# Autodesk Inventor assembly: a
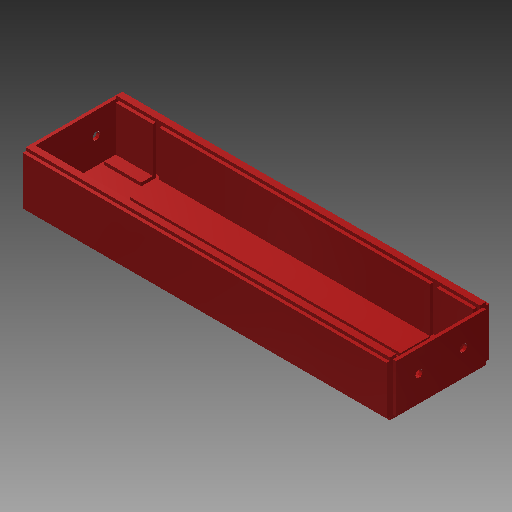
[picture p0: Inventor's stored thumbnail of the model, 512x512]
Saved by Autodesk Inventor 2017 (Build 210142000, 142)
## iProperties
Created: 2015-10-11
Part Number: a
Document SubType Name: Assembly
Designer: daniel
Author: daniel
## Documents named in this file (12)
- C:\Users\daniel\Documents\GitHub\cardboard-stage-metric\stage\a.iam
- C:\Users\daniel\Documents\GitHub\cardboard-stage-metric\stage\aa.ipt
- C:\Users\daniel\Documents\GitHub\cardboard-stage-metric\stage\ab.ipt
- C:\Users\daniel\Documents\GitHub\cardboard-stage-metric\stage\ac.ipt
- C:\Users\daniel\Documents\GitHub\cardboard-stage-metric\stage\ad.ipt
- C:\Users\daniel\Documents\GitHub\cardboard-stage-metric\stage\ae.ipt
- C:\Users\daniel\Documents\GitHub\cardboard-stage-metric\stage\af.ipt
- C:\Users\daniel\Documents\GitHub\cardboard-stage-metric\stage\ah.ipt
- C:\Users\daniel\Documents\GitHub\cardboard-stage-metric\stage\ai.ipt
- C:\Users\daniel\Documents\GitHub\cardboard-stage-metric\stage\base.ipt
- C:\Users\daniel\Documents\GitHub\cardboard-stage-metric\stage\aj.ipt
- C:\Users\daniel\Documents\GitHub\cardboard-stage-metric\stage\ak.ipt
## Components (23 placed, 10 different names)
1. aa:1 — Mate:5, Mate:6, Flush:1, Flush:2, Mate:7, Mate:8, Flush:4, Mate:21, Mate:22, Mate:23
2. ab:1 — Flush:19, Flush:20, Mate:21, Mate:22
3. ac:1 — Flush:19, Flush:20, Mate:23, Mate:24, Flush:24, Mate:26
4. ad:1 — Mate:5, Mate:6, Flush:1, Mate:9, Mate:10, Mate:15
5. ae:1 — Flush:3, Mate:9, Mate:10, Flush:4, Flush:5, Mate:19
6. af:1 — Mate:16, Flush:12, Flush:16, Mate:19, Flush:33, Flush:38, Flush:44, Flush:45
7. ah:1 — Mate:16, Flush:12, Flush:34, Flush:36, Flush:38
8. ad:2 — Flush:2, Mate:7, Mate:8, Mate:11, Flush:7, Flush:37
9. ae:2 — Flush:3, Flush:5, Mate:11, Mate:18, Mate:20, Flush:18
10. ai:1 — Flush:6, Flush:7, Mate:24, Flush:26
11. ai:2 — Flush:6, Mate:15, Mate:25, Flush:23, Flush:24, Flush:25, Mate:26
12. af:2 — Flush:16, Mate:18, Mate:20, Flush:18, Flush:32, Flush:46
13. ah:2 — Flush:36, Flush:47
14. ai:3 — Flush:21, Flush:22, Mate:25, Flush:26
15. ai:4 — Flush:21, Flush:22, Flush:23, Flush:25
16. af:3 — Flush:33
17. ah:3 — Flush:34, Flush:35, Flush:48, Mate:30
18. af:4 — Flush:32
19. ah:4 — Flush:35, Flush:37
20. aj:1 — Flush:39, Flush:42, Flush:43, Flush:46
21. ak:1 — Flush:42, Flush:43, Flush:47, Flush:49
22. aj:2 — Flush:39, Flush:41, Flush:44, Flush:45, Mate:29
23. ak:2 — Flush:41, Mate:29, Flush:48, Mate:30, Flush:49
## Relationships (65: Flush 42, Mate 23)
- Mate:5: aa:1 ↔ ad:1
- Mate:6: aa:1 ↔ ad:1
- Flush:1: aa:1 ↔ ad:1
- Flush:2: aa:1 ↔ ad:2
- Mate:7: aa:1 ↔ ad:2
- Mate:8: aa:1 ↔ ad:2
- Flush:3: ae:1 ↔ ae:2
- Mate:9: ad:1 ↔ ae:1
- Mate:10: ad:1 ↔ ae:1
- Flush:4: aa:1 ↔ ae:1
- Flush:5: ae:1 ↔ ae:2
- Mate:11: ad:2 ↔ ae:2
- Flush:6: ai:1 ↔ ai:2
- Flush:7: ad:2 ↔ ai:1
- Mate:15: ad:1 ↔ ai:2
- Mate:16: af:1 ↔ ah:1
- Flush:12: af:1 ↔ ah:1
- [Mate]: af:2 ↔ ah:2
- [Flush]: af:2 ↔ ah:2
- [Flush]: af:2 ↔ ah:2
- Flush:16: af:1 ↔ af:2
- Mate:19: ae:1 ↔ af:1
- Mate:18: ae:2 ↔ af:2
- Mate:20: ae:2 ↔ af:2
- Flush:18 (-4.3 mm): ae:2 ↔ af:2
- Flush:19: ab:1 ↔ ac:1
- Flush:20: ab:1 ↔ ac:1
- Mate:21: aa:1 ↔ ab:1
- Mate:22: aa:1 ↔ ab:1
- Mate:23: aa:1 ↔ ac:1
- Mate:24: ac:1 ↔ ai:1
- Flush:21: ai:3 ↔ ai:4
- Flush:22: ai:3 ↔ ai:4
- Mate:25: ai:2 ↔ ai:3
- Flush:23: ai:2 ↔ ai:4
- Flush:24: ac:1 ↔ ai:2
- Flush:25: ai:2 ↔ ai:4
- Flush:26: ai:1 ↔ ai:3
- Mate:26: ac:1 ↔ ai:2
- [Mate]: af:3 ↔ ah:3
- [Flush]: af:3 ↔ ah:3
- [Flush]: af:3 ↔ ah:3
- [Mate]: af:4 ↔ ah:4
- [Flush]: af:4 ↔ ah:4
- [Flush]: af:4 ↔ ah:4
- [Flush]: af:3 ↔ af:4
- Flush:32: af:2 ↔ af:4
- Flush:33: af:1 ↔ af:3
- Flush:34: ah:1 ↔ ah:3
- Flush:35: ah:3 ↔ ah:4
- Flush:36: ah:1 ↔ ah:2
- Flush:37 (4.3 mm): ad:2 ↔ ah:4
- Flush:38: af:1 ↔ ah:1
- Flush:39: aj:1 ↔ aj:2
- Flush:41: aj:2 ↔ ak:2
- Flush:42: aj:1 ↔ ak:1
- Flush:43: aj:1 ↔ ak:1
- Flush:44: af:1 ↔ aj:2
- Flush:45: af:1 ↔ aj:2
- Flush:46: af:2 ↔ aj:1
- Mate:29: aj:2 ↔ ak:2
- Flush:47: ah:2 ↔ ak:1
- Flush:48: ah:3 ↔ ak:2
- Mate:30 (8.6 mm): ah:3 ↔ ak:2
- Flush:49: ak:1 ↔ ak:2
## Named parameters: d28_d25 = 0 mm, d29_d26 = 0 mm, d30_d27 = 0 mm, d52_d25 = 0 mm, d53_d26 = 0 mm, d54_d27 = 0 mm, d55_d28_d25 = 0 mm, d56_d29_d26 = 0 mm, d57_d30_d27 = 0 mm, d58_d32 = 0 mm, material_thickness = 4.3 mm
